# Autodesk Inventor assembly: Assembly3
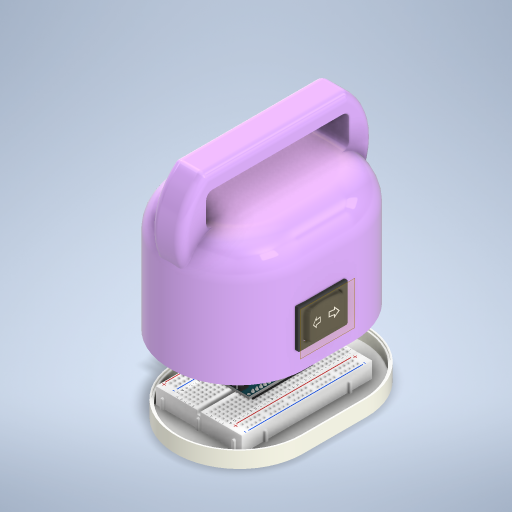
[picture p0: Inventor's stored thumbnail of the model, 512x512]
Saved by Autodesk Inventor 2024 (Build 280153000, 153)
## iProperties
Created: 2024-05-30
Part Number: Assembly3
Document SubType Name: Assembly
Designer: Andre
Author: Andre
## Documents named in this file (8)
- C:\Users\Andre\Downloads\funbioo\Assembly3.iam
- C:\Users\Andre\OneDrive\Escritorio\funbioo\cuerpo.ipt
- C:\Users\Andre\OneDrive\Escritorio\funbioo\tapa.ipt
- C:\Users\Andre\Downloads\arduino-nano-7.snapshot.2 (1)\arduino nano\arduino nano.ipt
- C:\Users\Andre\Downloads\flexible-printed-sensor-1.snapshot.1\FlexiblePrintedSensor\FlexiblePrintedSensor.ipt
- C:\Users\Andre\Downloads\FUNBIO\FUNBIO\clear-5mm-led-light-1.snapshot.7\Clear LED.ipt
- C:\Users\Andre\Downloads\rs223-4c-1.snapshot.1 (1)\Переключатель клавишный, контакты 6T, 35А, 12В, ( ON)-OFF-(ON ), RS223-4C\Переключатель клавишный, контакты 6T, 35А, 12В, ( ON)-OFF-(ON ), RS223-4C.ipt
- C:\Users\Andre\Downloads\protoboard-400-pts-1.snapshot.5\proto_400\proto_400.ipt
## Components (11 placed, 7 different names)
1. cuerpo:1 — Mate:1, Mate:2, Mate:3, Mate:4
2. tapa:1
3. arduino nano:1
4. FlexiblePrintedSensor:2
5. FlexiblePrintedSensor:3
6. Clear LED:1 — Mate:1
7. Clear LED:2 — Mate:2
8. Clear LED:3 — Mate:3
9. Clear LED:4 — Mate:4
10. Переключатель клавишный, контакты 6T, 35А, 12В, ( ON)-OFF-(ON ), RS223-4C:2
11. proto_400:2
## Relationships (4: Mate 4)
- Mate:1: cuerpo:1 ↔ Clear LED:1
- Mate:2: cuerpo:1 ↔ Clear LED:2
- Mate:3: cuerpo:1 ↔ Clear LED:3
- Mate:4: cuerpo:1 ↔ Clear LED:4
